# Autodesk Inventor assembly: mainASM
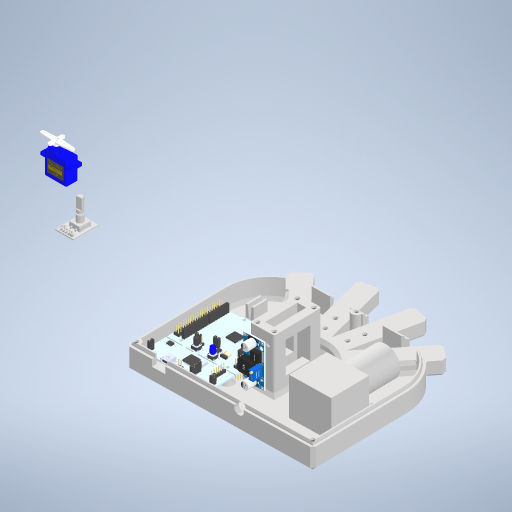
[picture p0: Inventor's stored thumbnail of the model, 512x512]
Saved by Autodesk Inventor 2024.2 (Build 282272000, 272)
## iProperties
Created: 2024-03-11
Part Number: mainASM
Document SubType Name: Assembly
Designer: Daniel
Author: Daniel
## Documents named in this file (7)
- C:\Users\Daniel\Desktop\pmik_2024l_jd\mechanical\mainASM.iam
- C:\Users\Daniel\Desktop\pmik_2024l_jd\mechanical\STEPS\NUCLEO-F091RC.iam
- C:\Users\Daniel\Desktop\pmik_2024l_jd\mechanical\STEPS\SG90 - Micro Servo 9g - Tower Pro.iam
- C:\Users\Daniel\Desktop\pmik_2024l_jd\mechanical\STEPS\KY-040 Rotary Encoder.iam
- C:\Users\Daniel\Desktop\pmik_2024l_jd\mechanical\bottom.ipt
- C:\Users\Daniel\Desktop\pmik_2024l_jd\mechanical\Pump.ipt
- C:\Users\Daniel\Desktop\pmik_2024l_jd\mechanical\STEPS\LM2596 DC to DC Buck Converter 3 A.iam
## Components (6 placed, 6 different names)
1. NUCLEO-F091RC:1 [sub-assembly] — Zestawiające:3, Zestawiające:4, Zestawiające:5
2. SG90 - Micro Servo 9g - Tower Pro:1 [sub-assembly]
3. KY-040 Rotary Encoder:1 [sub-assembly]
4. bottom:1 — Równoległe:1, Kątowe:1, Zestawiające:3, Zestawiające:4, Zestawiające:5, Zestawiające:6, Zestawiające:7, Zestawiające:8, Zestawiające:9, Równoległe:2, Równoległe:3
5. Pump:1 — Kątowe:1, Zestawiające:6, Zestawiające:7, Zestawiające:8
6. LM2596 DC to DC Buck Converter 3 A:1 [sub-assembly] — Zestawiające:9, Równoległe:2, Równoległe:3
## Relationships (11: Mate 7, Flush 3, Angle 1)
- Równoległe:1 [Flush]: bottom:1
- Kątowe:1 [Angle] (180 deg): bottom:1 ↔ Pump:1
- Zestawiające:3 [Mate] (3 mm): NUCLEO-F091RC:1 ↔ bottom:1
- Zestawiające:4 [Mate] (2 mm): NUCLEO-F091RC:1 ↔ bottom:1
- Zestawiające:5 [Mate] (5 mm): NUCLEO-F091RC:1 ↔ bottom:1
- Zestawiające:6 [Mate] (25 mm): bottom:1 ↔ Pump:1
- Zestawiające:7 [Mate] (5 mm): bottom:1 ↔ Pump:1
- Zestawiające:8 [Mate] (3 mm): bottom:1 ↔ Pump:1
- Zestawiające:9 [Mate] (5 mm): bottom:1 ↔ LM2596 DC to DC Buck Converter 3 A:1
- Równoległe:2 [Flush] (5 mm): bottom:1 ↔ LM2596 DC to DC Buck Converter 3 A:1
- Równoległe:3 [Flush] (4 mm): bottom:1 ↔ LM2596 DC to DC Buck Converter 3 A:1
